# Autodesk Inventor assembly: black-suspension
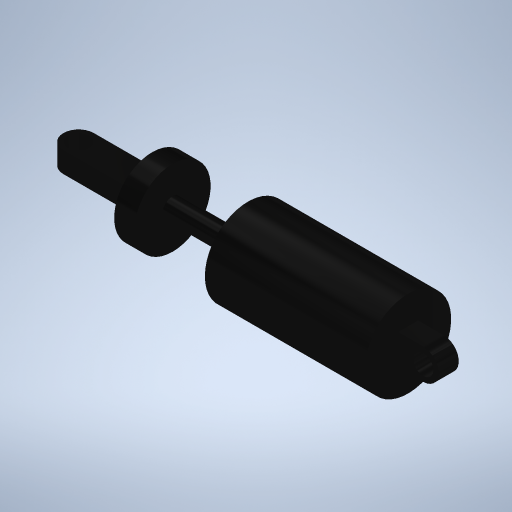
[picture p0: Inventor's stored thumbnail of the model, 512x512]
Saved by Autodesk Inventor 2024.1 (Build 281209000, 209)
## iProperties
Created: 2023-11-21
Part Number: black-suspension
Document SubType Name: Assembly
Designer: haruy
Author: haruy
## Documents named in this file (3)
- C:\Users\haruy\OneDrive - Kyushu University\KURT_工房共有\2023~2024\ハード\CAD\2024NHK\000_parts\サスペンション\black-suspension.iam
- C:\Users\haruy\OneDrive - Kyushu University\KURT_工房共有\2023~2024\ハード\CAD\2024NHK\000_parts\サスペンション\black-suspension-top.ipt
- C:\Users\haruy\OneDrive - Kyushu University\KURT_工房共有\2023~2024\ハード\CAD\2024NHK\000_parts\サスペンション\black-suspension-under.ipt
## Components (2 placed, 2 different names)
1. black-suspension-top:1 — 円柱状:1, 角度:1
2. black-suspension-under:1 — 円柱状:1, 角度:1
## Relationships (2: CylindricalJoint 1, Angle 1)
- 円柱状:1 [CylindricalJoint]: black-suspension-top:1 ↔ black-suspension-under:1
- 角度:1 [Angle] (90 deg): black-suspension-top:1 ↔ black-suspension-under:1
